# Autodesk Inventor assembly: Linear actuator v12
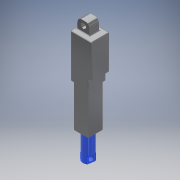
[picture p0: Inventor's stored thumbnail of the model, 180x180]
Saved by Autodesk Inventor 2019 (Build 230136000, 136)
## iProperties
Created: 2019-11-26
Part Number: Linear actuator v12
Document SubType Name: Assembly
Designer: Administrator
Title: Linear actuator v12 (3)
Author: Administrator
## Documents named in this file (3)
- C:\Users\wojta\Documents\Inventor\Reka\serwo\Linear actuator v12.iam
- C:\Users\wojta\Documents\Inventor\Reka\serwo\Body serwo.ipt
- C:\Users\wojta\Documents\Inventor\Reka\serwo\Push Rod.ipt
## Components (2 placed, 2 different names)
1. Body (3):1 — Zestawiający:1
2. Push Rod (3):1 — Zestawiający:1
## Relationships (1: Mate 1)
- Zestawiający:1 [Mate]: Body (3):1 ↔ Push Rod (3):1
